# Autodesk Inventor assembly: Почти готово
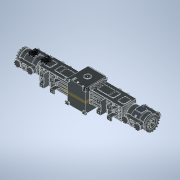
[picture p0: Inventor's stored thumbnail of the model, 180x180]
Saved by Autodesk Inventor 2021 (Build 250183000, 183)
## iProperties
Created: 2020-12-08
Part Number: Почти готово
Document SubType Name: Assembly
Designer: Тимоха
Author: Тимоха
## Documents named in this file (36)
- C:\Users\Тимоха\Desktop\КР Компрессор\compressor\Почти готово.iam
- C:\Users\Тимоха\Desktop\КР Компрессор\compressor\Картер.ipt
- C:\Users\Тимоха\Documents\Inventor\Content Center Files\R2021\ru-RU\Nut GOST 15524-70\Гайка M24-6H ГОСТ 15524-70.ipt
- C:\Users\Тимоха\Documents\Inventor\Content Center Files\R2021\ru-RU\GOST 11371-78  A\Шайба 27 ГОСТ 11371-78.ipt
- C:\Users\Тимоха\Desktop\КР Компрессор\compressor\Почти готово_CPY.iam
- C:\Users\Тимоха\Desktop\КР Компрессор\compressor\Вал.ipt
- C:\Users\Тимоха\Desktop\КР Компрессор\compressor\Нижняя часть коренного подшипника.ipt
- C:\Users\Тимоха\Desktop\КР Компрессор\compressor\Крышка коренного подшипника1.ipt
- C:\Users\Тимоха\Documents\Inventor\Content Center Files\R2021\ru-RU\Stud GOST 22038-76\Шпилька M24-6g×110 ГОСТ 22038-76.ipt
- C:\Users\Тимоха\Desktop\КР Компрессор\compressor\Под шатун.ipt
- C:\Users\Тимоха\Desktop\КР Компрессор\compressor\Шатун.ipt
- C:\Users\Тимоха\Desktop\КР Компрессор\compressor\Крышка стенки картера верх.ipt
- C:\Users\Тимоха\Desktop\КР Компрессор\compressor\Крышка стенки картера низ.ipt
- C:\Users\Тимоха\Desktop\КР Компрессор\compressor\Балка.ipt
- C:\Users\Тимоха\Documents\Inventor\Content Center Files\R2021\ru-RU\Bolt GOST R 50274-92\Болт M8-6g×16-F ГОСТ Р 50274-92.ipt
- C:\Users\Тимоха\Documents\Inventor\Content Center Files\R2021\ru-RU\Bolt GOST R 50274-92\Болт M8-6g×20-F ГОСТ Р 50274-92.ipt
- C:\Users\Тимоха\Desktop\КР Компрессор\compressor\Крышка картера 1.ipt
- C:\Users\Тимоха\Desktop\КР Компрессор\compressor\Крышка картера 2.ipt
- C:\Users\Тимоха\Desktop\КР Компрессор\compressor\Крышка картера 3.ipt
- C:\Users\Тимоха\Desktop\КР Компрессор\compressor\Крышка картера 4.ipt
- C:\Users\Тимоха\Desktop\КР Компрессор\compressor\Стяжка.ipt
- C:\Users\Тимоха\Documents\Inventor\Content Center Files\R2021\ru-RU\Nut GOST ISO 4034-2014\ГайкаM14ГОСТ ISO 4034-2014.ipt
- C:\Users\Тимоха\Desktop\КР Компрессор\compressor\Под стяжку.ipt
- C:\Users\Тимоха\Desktop\КР Компрессор\compressor\Под стяжку_MIR.ipt
- C:\Users\Тимоха\Desktop\КР Компрессор\compressor\Стяжка_MIR.ipt
- C:\Users\Тимоха\Desktop\КР Компрессор\compressor\Под стяжку_MIR1.ipt
- C:\Users\Тимоха\Desktop\КР Компрессор\compressor\Под стяжку_MIR_MIR.ipt
- C:\Users\Тимоха\Documents\Стекло.ipt
- C:\Users\Тимоха\Documents\Inventor\Content Center Files\R2021\ru-RU\GOST 7805-70\Болт M4-6gx10 ГОСТ 7805-70.ipt
- C:\Users\Тимоха\Desktop\КР Компрессор\compressor\Верхняя часть коренного подшипника.ipt
- C:\Users\Тимоха\Documents\Inventor\Content Center Files\R2021\ru-RU\GOST 7805-70\Болт M6-6gx40 ГОСТ 7805-70.ipt
- C:\Users\Тимоха\Documents\Inventor\Content Center Files\R2021\ru-RU\Nut GOST 15524-70\Гайка M6-6H ГОСТ 15524-70.ipt
- C:\Users\Тимоха\Desktop\КР Компрессор\compressor\Резина.ipt
- C:\Users\Тимоха\Desktop\КР Компрессор\compressor\Болт шатуна.ipt
- C:\Users\Тимоха\Documents\Inventor\Content Center Files\R2021\ru-RU\GOST 5918-73 (2)\Гайка 2 M39-6H ГОСТ 5918-73.ipt
- C:\Users\Тимоха\Desktop\КР Компрессор\compressor\Сапун.ipt
## Components (171 placed, 35 different names)
1. Картер:1 — Жесткий:407, Жесткий:410, Жесткий:411, Жесткий:412, Жесткий:421, Жесткий:422, Жесткий:423, Жесткий:428, Жесткий:429, Жесткий:431, Жесткий:433, Жесткий:434, Заподлицо:1, Заподлицо:2, Заподлицо:3, Заподлицо:4, Заподлицо:5, Заподлицо:6, Заподлицо:7, Заподлицо:8, Заподлицо:9, Жесткий:483, Жесткий:484, Заподлицо:14, Заподлицо:15, Заподлицо:16, Заподлицо:17, Заподлицо:18, Жесткий:560
2. Вал:1 — Жесткий:426, Совмещение:1, Жесткий:430, С поворотом:4
3. Нижняя часть коренного подшипника:2 — Жесткий:407, Жесткий:409
4. Нижняя часть коренного подшипника:3 — Жесткий:409
5. Крышка коренного подшипника1:1 — Жесткий:410
6. Крышка коренного подшипника1:2 — Жесткий:411, Совмещение:1
7. Шпилька ГОСТ 22038-76 M24-6g×110:1 — Жесткий:412, Жесткий:413, Жесткий:414
8. Гайка ГОСТ 15524-70 M24:54 — Жесткий:414
9. Шайба  ГОСТ 11371-78 28:22 — Жесткий:413
10. Шпилька ГОСТ 22038-76 M24-6g×110:2 — Жесткий:421
11. Гайка ГОСТ 15524-70 M24:55
12. Шайба  ГОСТ 11371-78 28:23
13. Шпилька ГОСТ 22038-76 M24-6g×110:3 — Жесткий:423
14. Гайка ГОСТ 15524-70 M24:56
15. Шайба  ГОСТ 11371-78 28:24
16. Шпилька ГОСТ 22038-76 M24-6g×110:4 — Жесткий:422
17. Гайка ГОСТ 15524-70 M24:57
18. Шайба  ГОСТ 11371-78 28:25
19. Под шатун:1 — Жесткий:425
20. Под шатун:2 — Жесткий:425, Жесткий:430
21. Под шатун:3 — Жесткий:426, Жесткий:427
22. Под шатун:4 — Жесткий:427, Цилиндрический:5
23. Почти готово_CPY:1 [sub-assembly] — Жесткий:429, С поворотом:5
24. Почти готово_CPY:2 [sub-assembly] — Жесткий:428, С поворотом:2, Заподлицо:7
25. Шатун:2 — Цилиндрический:5, С поворотом:2, Жесткий:574, Жесткий:575
26. Крышка стенки картера верх:1 — Жесткий:432, Жесткий:435, Жесткий:436, Жесткий:437, Жесткий:438, Жесткий:439, Жесткий:440, Жесткий:442, Жесткий:443, Жесткий:444, Жесткий:445, Жесткий:446, Жесткий:452, Жесткий:453, Жесткий:454, Жесткий:455, Жесткий:456, Жесткий:457, Жесткий:458, Жесткий:562, Жесткий:563, Жесткий:564, Жесткий:565, С поворотом:6
27. Крышка стенки картера низ:1 — Жесткий:431, Жесткий:432, Жесткий:447, Жесткий:448, Жесткий:449, Жесткий:450, Жесткий:451, Жесткий:566, Жесткий:567, Жесткий:568, Жесткий:569
28. Балка:1 — Жесткий:433
29. Балка:2 — Жесткий:434
30. Болт ГОСТ Р 50274-92 M8-6g×20-F:1 — Жесткий:435
31. Болт ГОСТ Р 50274-92 M8-6g×16-F:1 — Жесткий:439
32. Болт ГОСТ Р 50274-92 M8-6g×16-F:2 — Жесткий:436
33. Болт ГОСТ Р 50274-92 M8-6g×16-F:3 — Жесткий:440
34. Болт ГОСТ Р 50274-92 M8-6g×16-F:5 — Жесткий:438
35. Болт ГОСТ Р 50274-92 M8-6g×16-F:6 — Жесткий:442
36. Болт ГОСТ Р 50274-92 M8-6g×16-F:7 — Жесткий:437
37. Болт ГОСТ Р 50274-92 M8-6g×20-F:2 — Жесткий:443
38. Болт ГОСТ Р 50274-92 M8-6g×16-F:8 — Жесткий:446
39. Болт ГОСТ Р 50274-92 M8-6g×16-F:9 — Жесткий:444
40. Болт ГОСТ Р 50274-92 M8-6g×16-F:10 — Жесткий:450
41. Болт ГОСТ Р 50274-92 M8-6g×16-F:11 — Жесткий:451
42. Болт ГОСТ Р 50274-92 M8-6g×16-F:12 — Жесткий:445
43. Болт ГОСТ Р 50274-92 M8-6g×16-F:13 — Жесткий:447
44. Болт ГОСТ Р 50274-92 M8-6g×16-F:14 — Жесткий:449
45. Болт ГОСТ Р 50274-92 M8-6g×20-F:3 — Жесткий:452
46. Болт ГОСТ Р 50274-92 M8-6g×16-F:19 — Жесткий:448
47. Крышка картера 1:1 — Заподлицо:1, Заподлицо:2, Жесткий:459, Жесткий:460, Жесткий:461, Заподлицо:10, Жесткий:470, Жесткий:471, Жесткий:472, Жесткий:473, Жесткий:474, Жесткий:475, Жесткий:476
48. Крышка картера 2:1 — Заподлицо:3, Заподлицо:4, Жесткий:462, Жесткий:463, Жесткий:464, С поворотом:3, Жесткий:465, Жесткий:466, Жесткий:467, Заподлицо:11, Заподлицо:12, Жесткий:578
49. Крышка картера 3:1 — Заподлицо:5, Заподлицо:6, Жесткий:468, Жесткий:469, Заподлицо:13
50. Крышка картера 4:1 — Заподлицо:8, Заподлицо:9, Жесткий:477, Жесткий:478, Жесткий:479, Жесткий:480, Жесткий:481, Жесткий:482
51. Болт ГОСТ Р 50274-92 M8-6g×20-F:4 — Жесткий:453
52. Болт ГОСТ Р 50274-92 M8-6g×20-F:12 — Жесткий:471
53. Болт ГОСТ Р 50274-92 M8-6g×20-F:13 — Жесткий:473
54. Болт ГОСТ Р 50274-92 M8-6g×20-F:19 — Жесткий:468
55. Болт ГОСТ Р 50274-92 M8-6g×20-F:20 — Жесткий:469
56. Болт ГОСТ Р 50274-92 M8-6g×20-F:21 — Жесткий:460
57. Болт ГОСТ Р 50274-92 M8-6g×20-F:26 — Жесткий:454
58. Болт ГОСТ Р 50274-92 M8-6g×20-F:27 — Жесткий:463
59. Болт ГОСТ Р 50274-92 M8-6g×20-F:28 — Жесткий:462
60. Болт ГОСТ Р 50274-92 M8-6g×20-F:29 — Жесткий:458
61. Болт ГОСТ Р 50274-92 M8-6g×20-F:30 — Жесткий:465
62. Болт ГОСТ Р 50274-92 M8-6g×20-F:31 — Жесткий:466
63. Болт ГОСТ Р 50274-92 M8-6g×20-F:32 — Жесткий:467
64. Болт ГОСТ Р 50274-92 M8-6g×20-F:33 — Жесткий:455
65. Болт ГОСТ Р 50274-92 M8-6g×20-F:34 — Жесткий:456
66. Болт ГОСТ Р 50274-92 M8-6g×20-F:35 — Жесткий:457
67. Болт ГОСТ Р 50274-92 M8-6g×20-F:36 — Жесткий:461
68. Болт ГОСТ Р 50274-92 M8-6g×20-F:37 — Жесткий:459
69. Болт ГОСТ Р 50274-92 M8-6g×20-F:38 — Жесткий:464
70. Болт ГОСТ Р 50274-92 M8-6g×20-F:39 — С поворотом:3
71. Болт ГОСТ Р 50274-92 M8-6g×20-F:40 — Жесткий:470
72. Болт ГОСТ Р 50274-92 M8-6g×20-F:41 — Жесткий:472
73. Болт ГОСТ Р 50274-92 M8-6g×20-F:42 — Жесткий:474
74. Болт ГОСТ Р 50274-92 M8-6g×20-F:43 — Жесткий:475
75. Болт ГОСТ Р 50274-92 M8-6g×20-F:45 — Жесткий:476
76. Болт ГОСТ Р 50274-92 M8-6g×20-F:47
77. Болт ГОСТ Р 50274-92 M8-6g×20-F:48
78. Болт ГОСТ Р 50274-92 M8-6g×20-F:49
79. Болт ГОСТ Р 50274-92 M8-6g×20-F:50
80. Болт ГОСТ Р 50274-92 M8-6g×20-F:51
81. Болт ГОСТ Р 50274-92 M8-6g×20-F:52
82. Болт ГОСТ Р 50274-92 M8-6g×20-F:53
83. Болт ГОСТ Р 50274-92 M8-6g×20-F:54
84. Болт ГОСТ Р 50274-92 M8-6g×20-F:55
85. Болт ГОСТ Р 50274-92 M8-6g×20-F:56
86. Болт ГОСТ Р 50274-92 M8-6g×20-F:57
87. Болт ГОСТ Р 50274-92 M8-6g×20-F:58
88. Болт ГОСТ Р 50274-92 M8-6g×20-F:59
89. Болт ГОСТ Р 50274-92 M8-6g×20-F:60
90. Болт ГОСТ Р 50274-92 M8-6g×20-F:61
91. Болт ГОСТ Р 50274-92 M8-6g×20-F:62
92. Болт ГОСТ Р 50274-92 M8-6g×20-F:63
93. Болт ГОСТ Р 50274-92 M8-6g×20-F:64
94. Болт ГОСТ Р 50274-92 M8-6g×20-F:65
95. Болт ГОСТ Р 50274-92 M8-6g×20-F:66
96. Болт ГОСТ Р 50274-92 M8-6g×20-F:67
97. Болт ГОСТ Р 50274-92 M8-6g×20-F:68
98. Болт ГОСТ Р 50274-92 M8-6g×20-F:69
99. Болт ГОСТ Р 50274-92 M8-6g×20-F:70
100. Болт ГОСТ Р 50274-92 M8-6g×20-F:71
101. Болт ГОСТ Р 50274-92 M8-6g×20-F:72
102. Болт ГОСТ Р 50274-92 M8-6g×20-F:73
103. Болт ГОСТ Р 50274-92 M8-6g×20-F:74
104. Болт ГОСТ Р 50274-92 M8-6g×20-F:75
105. Болт ГОСТ Р 50274-92 M8-6g×20-F:76
106. Болт ГОСТ Р 50274-92 M8-6g×20-F:77
107. Болт ГОСТ Р 50274-92 M8-6g×20-F:78
108. Болт ГОСТ Р 50274-92 M8-6g×20-F:79
109. Болт ГОСТ Р 50274-92 M8-6g×20-F:80
110. Болт ГОСТ Р 50274-92 M8-6g×20-F:81
111. Болт ГОСТ Р 50274-92 M8-6g×20-F:82
112. Болт ГОСТ Р 50274-92 M8-6g×20-F:83
113. Болт ГОСТ Р 50274-92 M8-6g×20-F:84
114. Болт ГОСТ Р 50274-92 M8-6g×20-F:85
115. Болт ГОСТ Р 50274-92 M8-6g×20-F:86
116. Болт ГОСТ Р 50274-92 M8-6g×20-F:87 — Жесткий:477
117. Болт ГОСТ Р 50274-92 M8-6g×20-F:88 — Жесткий:478
118. Болт ГОСТ Р 50274-92 M8-6g×20-F:89 — Жесткий:480
119. Болт ГОСТ Р 50274-92 M8-6g×20-F:90 — Жесткий:481
120. Болт ГОСТ Р 50274-92 M8-6g×20-F:91 — Жесткий:479
121. Болт ГОСТ Р 50274-92 M8-6g×20-F:92 — Жесткий:482
122. Стяжка:1 — Жесткий:483
123. Гайка ГОСТ ISO 4034-2014 (M14):1 — Жесткий:485
124. Стяжка:2 — Жесткий:484
125. Под стяжку:1 — Заподлицо:14, Заподлицо:15, Жесткий:485, Жесткий:486
126. Гайка ГОСТ ISO 4034-2014 (M14):2 — Жесткий:486
127. Гайка ГОСТ ISO 4034-2014 (M14):3 — Жесткий:487
128. Под стяжку_MIR:1 — Жесткий:487, Жесткий:488
129. Гайка ГОСТ ISO 4034-2014 (M14):4 — Жесткий:488
130. Стяжка_MIR:1
131. Гайка ГОСТ ISO 4034-2014 (M14):5 — Жесткий:489
132. Стяжка_MIR:2
133. Под стяжку_MIR1:1 — Жесткий:489, Жесткий:490
134. Гайка ГОСТ ISO 4034-2014 (M14):6 — Жесткий:490
135. Гайка ГОСТ ISO 4034-2014 (M14):7 — Жесткий:491
136. Под стяжку_MIR_MIR:1 — Жесткий:491, Жесткий:492
137. Гайка ГОСТ ISO 4034-2014 (M14):8 — Жесткий:492
138. Шатун:3 — С поворотом:4, С поворотом:5, Жесткий:570, Жесткий:572
139. Стекло:1 — Заподлицо:17, Заподлицо:18, Жесткий:548, Жесткий:549, Жесткий:550, Жесткий:551, Жесткий:552, Жесткий:553, Жесткий:554, Жесткий:555, Жесткий:556, Жесткий:557, Жесткий:558, Жесткий:559
140. Болт ГОСТ 7805-70 M4-6gx10:2 — Жесткий:549
141. Болт ГОСТ 7805-70 M4-6gx10:3 — Жесткий:552
142. Болт ГОСТ 7805-70 M4-6gx10:4 — Жесткий:554
143. Болт ГОСТ 7805-70 M4-6gx10:5 — Жесткий:550
144. Болт ГОСТ 7805-70 M4-6gx10:6 — Жесткий:548
145. Болт ГОСТ 7805-70 M4-6gx10:7 — Жесткий:551
146. Болт ГОСТ 7805-70 M4-6gx10:9 — Жесткий:559
147. Болт ГОСТ 7805-70 M4-6gx10:10 — Жесткий:556
148. Болт ГОСТ 7805-70 M4-6gx10:14 — Жесткий:553
149. Болт ГОСТ 7805-70 M4-6gx10:15 — Жесткий:555
150. Болт ГОСТ 7805-70 M4-6gx10:16 — Жесткий:557
151. Болт ГОСТ 7805-70 M4-6gx10:17 — Жесткий:558
152. Верхняя часть коренного подшипника:2 — Жесткий:560, Жесткий:561
153. Верхняя часть коренного подшипника:3 — Жесткий:561
154. Болт ГОСТ 7805-70 M6-6gx40:1 — Жесткий:562
155. Болт ГОСТ 7805-70 M6-6gx40:2 — Жесткий:565
156. Болт ГОСТ 7805-70 M6-6gx40:3 — Жесткий:564
157. Болт ГОСТ 7805-70 M6-6gx40:4 — Жесткий:563
158. Гайка ГОСТ 15524-70 M6:1 — Жесткий:566
159. Гайка ГОСТ 15524-70 M6:2 — Жесткий:567
160. Гайка ГОСТ 15524-70 M6:3 — Жесткий:568
161. Гайка ГОСТ 15524-70 M6:4 — Жесткий:569
162. Резина:1 — С поворотом:6
163. Болт шатуна:1 — Жесткий:572, Жесткий:573
164. Болт шатуна:2 — Жесткий:570, Жесткий:571
165. Болт шатуна:3 — Жесткий:575, Жесткий:577
166. Болт шатуна:4 — Жесткий:574, Жесткий:576
167. Гайка 2 ГОСТ 5918-73 M39:1 — Жесткий:571
168. Гайка 2 ГОСТ 5918-73 M39:2 — Жесткий:573
169. Гайка 2 ГОСТ 5918-73 M39:3 — Жесткий:576
170. Гайка 2 ГОСТ 5918-73 M39:4 — Жесткий:577
171. Сапун:1 — Жесткий:578
## Relationships (139: WeldJoint 114, Flush 18, RevoluteJoint 5, CylindricalJoint 1, Mate 1)
- Жесткий:407 [WeldJoint]: Картер:1 ↔ Нижняя часть коренного подшипника:2
- Жесткий:409 [WeldJoint]: Нижняя часть коренного подшипника:2 ↔ Нижняя часть коренного подшипника:3
- Жесткий:410 [WeldJoint]: Картер:1 ↔ Крышка коренного подшипника1:1
- Жесткий:411 [WeldJoint]: Картер:1 ↔ Крышка коренного подшипника1:2
- Жесткий:412 [WeldJoint]: Картер:1 ↔ Шпилька ГОСТ 22038-76 M24-6g×110:1
- Жесткий:413 [WeldJoint] (-35 mm): Шпилька ГОСТ 22038-76 M24-6g×110:1 ↔ Шайба  ГОСТ 11371-78 28:22
- Жесткий:414 [WeldJoint] (-5.75 mm): Шпилька ГОСТ 22038-76 M24-6g×110:1 ↔ Гайка ГОСТ 15524-70 M24:54
- [WeldJoint] (-35 mm): Шпилька ГОСТ 22038-76 M24-6g×110:2 ↔ Шайба  ГОСТ 11371-78 28:23
- [WeldJoint] (-5.75 mm): Шпилька ГОСТ 22038-76 M24-6g×110:2 ↔ Гайка ГОСТ 15524-70 M24:55
- [WeldJoint] (-35 mm): Шпилька ГОСТ 22038-76 M24-6g×110:3 ↔ Шайба  ГОСТ 11371-78 28:24
- [WeldJoint] (-5.75 mm): Шпилька ГОСТ 22038-76 M24-6g×110:3 ↔ Гайка ГОСТ 15524-70 M24:56
- [WeldJoint] (-35 mm): Шпилька ГОСТ 22038-76 M24-6g×110:4 ↔ Шайба  ГОСТ 11371-78 28:25
- [WeldJoint] (-5.75 mm): Шпилька ГОСТ 22038-76 M24-6g×110:4 ↔ Гайка ГОСТ 15524-70 M24:57
- Жесткий:421 [WeldJoint]: Картер:1 ↔ Шпилька ГОСТ 22038-76 M24-6g×110:2
- Жесткий:422 [WeldJoint]: Картер:1 ↔ Шпилька ГОСТ 22038-76 M24-6g×110:4
- Жесткий:423 [WeldJoint]: Картер:1 ↔ Шпилька ГОСТ 22038-76 M24-6g×110:3
- Жесткий:425 [WeldJoint]: Под шатун:1 ↔ Под шатун:2
- Жесткий:426 [WeldJoint]: Вал:1 ↔ Под шатун:3
- Жесткий:427 [WeldJoint]: Под шатун:3 ↔ Под шатун:4
- Жесткий:428 [WeldJoint]: Картер:1 ↔ Почти готово_CPY:2
- Жесткий:429 [WeldJoint]: Картер:1 ↔ Почти готово_CPY:1
- Цилиндрический:5 [CylindricalJoint]: Под шатун:4 ↔ Шатун:2
- С поворотом:2 [RevoluteJoint]: Почти готово_CPY:2 ↔ Шатун:2
- Совмещение:1 [Mate] (5 mm): Вал:1 ↔ Крышка коренного подшипника1:2
- Жесткий:430 [WeldJoint]: Вал:1 ↔ Под шатун:2
- Жесткий:431 [WeldJoint]: Картер:1 ↔ Крышка стенки картера низ:1
- Жесткий:432 [WeldJoint]: Крышка стенки картера верх:1 ↔ Крышка стенки картера низ:1
- Жесткий:433 [WeldJoint]: Картер:1 ↔ Балка:1
- Жесткий:434 [WeldJoint]: Картер:1 ↔ Балка:2
- Жесткий:435 [WeldJoint]: Крышка стенки картера верх:1 ↔ Болт ГОСТ Р 50274-92 M8-6g×20-F:1
- Жесткий:436 [WeldJoint]: Крышка стенки картера верх:1 ↔ Болт ГОСТ Р 50274-92 M8-6g×16-F:2
- Жесткий:437 [WeldJoint]: Крышка стенки картера верх:1 ↔ Болт ГОСТ Р 50274-92 M8-6g×16-F:7
- Жесткий:438 [WeldJoint]: Крышка стенки картера верх:1 ↔ Болт ГОСТ Р 50274-92 M8-6g×16-F:5
- Жесткий:439 [WeldJoint]: Крышка стенки картера верх:1 ↔ Болт ГОСТ Р 50274-92 M8-6g×16-F:1
- Жесткий:440 [WeldJoint]: Крышка стенки картера верх:1 ↔ Болт ГОСТ Р 50274-92 M8-6g×16-F:3
- Жесткий:442 [WeldJoint]: Крышка стенки картера верх:1 ↔ Болт ГОСТ Р 50274-92 M8-6g×16-F:6
- Жесткий:443 [WeldJoint]: Крышка стенки картера верх:1 ↔ Болт ГОСТ Р 50274-92 M8-6g×20-F:2
- Жесткий:444 [WeldJoint]: Крышка стенки картера верх:1 ↔ Болт ГОСТ Р 50274-92 M8-6g×16-F:9
- Жесткий:445 [WeldJoint]: Крышка стенки картера верх:1 ↔ Болт ГОСТ Р 50274-92 M8-6g×16-F:12
- Жесткий:446 [WeldJoint]: Крышка стенки картера верх:1 ↔ Болт ГОСТ Р 50274-92 M8-6g×16-F:8
- Жесткий:447 [WeldJoint]: Крышка стенки картера низ:1 ↔ Болт ГОСТ Р 50274-92 M8-6g×16-F:13
- Жесткий:448 [WeldJoint]: Крышка стенки картера низ:1 ↔ Болт ГОСТ Р 50274-92 M8-6g×16-F:19
- Жесткий:449 [WeldJoint]: Крышка стенки картера низ:1 ↔ Болт ГОСТ Р 50274-92 M8-6g×16-F:14
- Жесткий:450 [WeldJoint]: Крышка стенки картера низ:1 ↔ Болт ГОСТ Р 50274-92 M8-6g×16-F:10
- Жесткий:451 [WeldJoint]: Крышка стенки картера низ:1 ↔ Болт ГОСТ Р 50274-92 M8-6g×16-F:11
- Жесткий:452 [WeldJoint]: Крышка стенки картера верх:1 ↔ Болт ГОСТ Р 50274-92 M8-6g×20-F:3
- Заподлицо:1 [Flush]: Картер:1 ↔ Крышка картера 1:1
- Заподлицо:2 [Flush]: Картер:1 ↔ Крышка картера 1:1
- Заподлицо:3 [Flush]: Картер:1 ↔ Крышка картера 2:1
- Заподлицо:4 [Flush]: Картер:1 ↔ Крышка картера 2:1
- Заподлицо:5 [Flush]: Картер:1 ↔ Крышка картера 3:1
- Заподлицо:6 [Flush]: Картер:1 ↔ Крышка картера 3:1
- Заподлицо:7 [Flush]: Картер:1 ↔ Почти готово_CPY:2
- Заподлицо:8 [Flush]: Картер:1 ↔ Крышка картера 4:1
- Заподлицо:9 [Flush]: Картер:1 ↔ Крышка картера 4:1
- Жесткий:453 [WeldJoint]: Крышка стенки картера верх:1 ↔ Болт ГОСТ Р 50274-92 M8-6g×20-F:4
- Жесткий:454 [WeldJoint]: Крышка стенки картера верх:1 ↔ Болт ГОСТ Р 50274-92 M8-6g×20-F:26
- Жесткий:455 [WeldJoint]: Крышка стенки картера верх:1 ↔ Болт ГОСТ Р 50274-92 M8-6g×20-F:33
- Жесткий:456 [WeldJoint]: Крышка стенки картера верх:1 ↔ Болт ГОСТ Р 50274-92 M8-6g×20-F:34
- Жесткий:457 [WeldJoint]: Крышка стенки картера верх:1 ↔ Болт ГОСТ Р 50274-92 M8-6g×20-F:35
- Жесткий:458 [WeldJoint]: Крышка стенки картера верх:1 ↔ Болт ГОСТ Р 50274-92 M8-6g×20-F:29
- Жесткий:459 [WeldJoint]: Крышка картера 1:1 ↔ Болт ГОСТ Р 50274-92 M8-6g×20-F:37
- Жесткий:460 [WeldJoint]: Крышка картера 1:1 ↔ Болт ГОСТ Р 50274-92 M8-6g×20-F:21
- Жесткий:461 [WeldJoint]: Крышка картера 1:1 ↔ Болт ГОСТ Р 50274-92 M8-6g×20-F:36
- Жесткий:462 [WeldJoint]: Крышка картера 2:1 ↔ Болт ГОСТ Р 50274-92 M8-6g×20-F:28
- Жесткий:463 [WeldJoint]: Крышка картера 2:1 ↔ Болт ГОСТ Р 50274-92 M8-6g×20-F:27
- Жесткий:464 [WeldJoint]: Крышка картера 2:1 ↔ Болт ГОСТ Р 50274-92 M8-6g×20-F:38
- С поворотом:3 [RevoluteJoint]: Крышка картера 2:1 ↔ Болт ГОСТ Р 50274-92 M8-6g×20-F:39
- Жесткий:465 [WeldJoint]: Крышка картера 2:1 ↔ Болт ГОСТ Р 50274-92 M8-6g×20-F:30
- Жесткий:466 [WeldJoint]: Крышка картера 2:1 ↔ Болт ГОСТ Р 50274-92 M8-6g×20-F:31
- Жесткий:467 [WeldJoint]: Крышка картера 2:1 ↔ Болт ГОСТ Р 50274-92 M8-6g×20-F:32
- Жесткий:468 [WeldJoint]: Крышка картера 3:1 ↔ Болт ГОСТ Р 50274-92 M8-6g×20-F:19
- Жесткий:469 [WeldJoint]: Крышка картера 3:1 ↔ Болт ГОСТ Р 50274-92 M8-6g×20-F:20
- Заподлицо:10 [Flush] (8 mm): Крышка картера 1:1
- Заподлицо:11 [Flush] (-326.9 mm): Крышка картера 2:1
- Заподлицо:12 [Flush] (8 mm): Крышка картера 2:1
- Заподлицо:13 [Flush] (-66.5 mm): Крышка картера 3:1
- Жесткий:470 [WeldJoint]: Крышка картера 1:1 ↔ Болт ГОСТ Р 50274-92 M8-6g×20-F:40
- Жесткий:471 [WeldJoint]: Крышка картера 1:1 ↔ Болт ГОСТ Р 50274-92 M8-6g×20-F:12
- Жесткий:472 [WeldJoint]: Крышка картера 1:1 ↔ Болт ГОСТ Р 50274-92 M8-6g×20-F:41
- Жесткий:473 [WeldJoint]: Крышка картера 1:1 ↔ Болт ГОСТ Р 50274-92 M8-6g×20-F:13
- Жесткий:474 [WeldJoint]: Крышка картера 1:1 ↔ Болт ГОСТ Р 50274-92 M8-6g×20-F:42
- Жесткий:475 [WeldJoint]: Крышка картера 1:1 ↔ Болт ГОСТ Р 50274-92 M8-6g×20-F:43
- Жесткий:476 [WeldJoint]: Крышка картера 1:1 ↔ Болт ГОСТ Р 50274-92 M8-6g×20-F:45
- Жесткий:477 [WeldJoint]: Крышка картера 4:1 ↔ Болт ГОСТ Р 50274-92 M8-6g×20-F:87
- Жесткий:478 [WeldJoint]: Крышка картера 4:1 ↔ Болт ГОСТ Р 50274-92 M8-6g×20-F:88
- Жесткий:479 [WeldJoint]: Крышка картера 4:1 ↔ Болт ГОСТ Р 50274-92 M8-6g×20-F:91
- Жесткий:480 [WeldJoint]: Крышка картера 4:1 ↔ Болт ГОСТ Р 50274-92 M8-6g×20-F:89
- Жесткий:481 [WeldJoint]: Крышка картера 4:1 ↔ Болт ГОСТ Р 50274-92 M8-6g×20-F:90
- Жесткий:482 [WeldJoint]: Крышка картера 4:1 ↔ Болт ГОСТ Р 50274-92 M8-6g×20-F:92
- Жесткий:483 [WeldJoint] (-40 mm): Картер:1 ↔ Стяжка:1
- Жесткий:484 [WeldJoint] (40 mm): Картер:1 ↔ Стяжка:2
- Заподлицо:14 [Flush]: Картер:1 ↔ Под стяжку:1
- Заподлицо:15 [Flush]: Картер:1 ↔ Под стяжку:1
- Жесткий:485 [WeldJoint]: Гайка ГОСТ ISO 4034-2014 (M14):1 ↔ Под стяжку:1
- Жесткий:486 [WeldJoint]: Под стяжку:1 ↔ Гайка ГОСТ ISO 4034-2014 (M14):2
- Жесткий:487 [WeldJoint]: Гайка ГОСТ ISO 4034-2014 (M14):3 ↔ Под стяжку_MIR:1
- Жесткий:488 [WeldJoint]: Под стяжку_MIR:1 ↔ Гайка ГОСТ ISO 4034-2014 (M14):4
- Заподлицо:16 [Flush] (-465 mm): Картер:1
- Жесткий:489 [WeldJoint]: Гайка ГОСТ ISO 4034-2014 (M14):5 ↔ Под стяжку_MIR1:1
- Жесткий:490 [WeldJoint]: Под стяжку_MIR1:1 ↔ Гайка ГОСТ ISO 4034-2014 (M14):6
- Жесткий:491 [WeldJoint]: Гайка ГОСТ ISO 4034-2014 (M14):7 ↔ Под стяжку_MIR_MIR:1
- Жесткий:492 [WeldJoint]: Под стяжку_MIR_MIR:1 ↔ Гайка ГОСТ ISO 4034-2014 (M14):8
- С поворотом:4 [RevoluteJoint]: Вал:1 ↔ Шатун:3
- С поворотом:5 [RevoluteJoint]: Почти готово_CPY:1 ↔ Шатун:3
- Заподлицо:17 [Flush]: Картер:1 ↔ Стекло:1
- Заподлицо:18 [Flush]: Картер:1 ↔ Стекло:1
- Жесткий:548 [WeldJoint]: Стекло:1 ↔ Болт ГОСТ 7805-70 M4-6gx10:6
- Жесткий:549 [WeldJoint]: Стекло:1 ↔ Болт ГОСТ 7805-70 M4-6gx10:2
- Жесткий:550 [WeldJoint]: Стекло:1 ↔ Болт ГОСТ 7805-70 M4-6gx10:5
- Жесткий:551 [WeldJoint]: Стекло:1 ↔ Болт ГОСТ 7805-70 M4-6gx10:7
- Жесткий:552 [WeldJoint]: Стекло:1 ↔ Болт ГОСТ 7805-70 M4-6gx10:3
- Жесткий:553 [WeldJoint]: Стекло:1 ↔ Болт ГОСТ 7805-70 M4-6gx10:14
- Жесткий:554 [WeldJoint]: Стекло:1 ↔ Болт ГОСТ 7805-70 M4-6gx10:4
- Жесткий:555 [WeldJoint]: Стекло:1 ↔ Болт ГОСТ 7805-70 M4-6gx10:15
- Жесткий:556 [WeldJoint]: Стекло:1 ↔ Болт ГОСТ 7805-70 M4-6gx10:10
- Жесткий:557 [WeldJoint]: Стекло:1 ↔ Болт ГОСТ 7805-70 M4-6gx10:16
- Жесткий:558 [WeldJoint]: Стекло:1 ↔ Болт ГОСТ 7805-70 M4-6gx10:17
- Жесткий:559 [WeldJoint]: Стекло:1 ↔ Болт ГОСТ 7805-70 M4-6gx10:9
- Жесткий:560 [WeldJoint]: Картер:1 ↔ Верхняя часть коренного подшипника:2
- Жесткий:561 [WeldJoint]: Верхняя часть коренного подшипника:2 ↔ Верхняя часть коренного подшипника:3
- Жесткий:562 [WeldJoint]: Крышка стенки картера верх:1 ↔ Болт ГОСТ 7805-70 M6-6gx40:1
- Жесткий:563 [WeldJoint]: Крышка стенки картера верх:1 ↔ Болт ГОСТ 7805-70 M6-6gx40:4
- Жесткий:564 [WeldJoint]: Крышка стенки картера верх:1 ↔ Болт ГОСТ 7805-70 M6-6gx40:3
- Жесткий:565 [WeldJoint]: Крышка стенки картера верх:1 ↔ Болт ГОСТ 7805-70 M6-6gx40:2
- Жесткий:566 [WeldJoint]: Крышка стенки картера низ:1 ↔ Гайка ГОСТ 15524-70 M6:1
- Жесткий:567 [WeldJoint]: Крышка стенки картера низ:1 ↔ Гайка ГОСТ 15524-70 M6:2
- Жесткий:568 [WeldJoint]: Крышка стенки картера низ:1 ↔ Гайка ГОСТ 15524-70 M6:3
- Жесткий:569 [WeldJoint]: Крышка стенки картера низ:1 ↔ Гайка ГОСТ 15524-70 M6:4
- С поворотом:6 [RevoluteJoint]: Крышка стенки картера верх:1 ↔ Резина:1
- Жесткий:570 [WeldJoint]: Шатун:3 ↔ Болт шатуна:2
- Жесткий:571 [WeldJoint] (-50 mm): Болт шатуна:2 ↔ Гайка 2 ГОСТ 5918-73 M39:1
- Жесткий:572 [WeldJoint]: Шатун:3 ↔ Болт шатуна:1
- Жесткий:573 [WeldJoint] (-50 mm): Болт шатуна:1 ↔ Гайка 2 ГОСТ 5918-73 M39:2
- Жесткий:574 [WeldJoint]: Шатун:2 ↔ Болт шатуна:4
- Жесткий:575 [WeldJoint]: Шатун:2 ↔ Болт шатуна:3
- Жесткий:576 [WeldJoint] (-50 mm): Болт шатуна:4 ↔ Гайка 2 ГОСТ 5918-73 M39:3
- Жесткий:577 [WeldJoint] (-50 mm): Болт шатуна:3 ↔ Гайка 2 ГОСТ 5918-73 M39:4
- Жесткий:578 [WeldJoint]: Крышка картера 2:1 ↔ Сапун:1
## Named parameters: d482_d480 = -35 mm, d483_d481 = -5.75 mm, d484_d480 = -35 mm, d485_d481 = -5.75 mm, d486_d480 = -35 mm, d487_d481 = -5.75 mm
